# Autodesk Inventor assembly: Exoskeleton
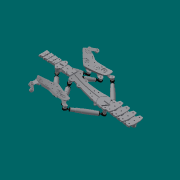
[picture p0: Inventor's stored thumbnail of the model, 180x180]
Saved by Autodesk Inventor 2015 SP1 (Build 190203100, 203)
## iProperties
Created: 2016-10-02
Part Number: Exoskeleton
Document SubType Name: Assembly
Designer: Val
Author: Val
## Documents named in this file (24)
- C:\Users\Val\Desktop\ExoGit\elysium-max-exoskeleton\src\Assemblies\Exoskeleton.iam
- C:\Users\Val\Desktop\ExoGit\elysium-max-exoskeleton\src\Assemblies\ChestDerived.iam
- C:\Users\Val\Desktop\ExoGit\elysium-max-exoskeleton\src\Assemblies\Spine.iam
- C:\Users\Val\Desktop\ExoGit\elysium-max-exoskeleton\src\Assemblies\Pelvis.iam
- C:\Users\Val\Desktop\ExoGit\elysium-max-exoskeleton\src\Assemblies\HipLeft.iam
- C:\Users\Val\Desktop\ExoGit\elysium-max-exoskeleton\src\Assemblies\HipRight.iam
- C:\Users\Val\Desktop\ExoGit\elysium-max-exoskeleton\src\Assemblies\ShoulderLeft.iam
- C:\Users\Val\Desktop\ExoGit\elysium-max-exoskeleton\src\Assemblies\ShoulderRight.iam
- C:\Users\Val\Desktop\ExoGit\elysium-max-exoskeleton\src\Assemblies\UpperArmLeft.iam
- C:\Users\Val\Desktop\ExoGit\elysium-max-exoskeleton\src\Assemblies\UpperArmRight.iam
- C:\Users\Val\Desktop\ExoGit\elysium-max-exoskeleton\src\Assemblies\ForearmLeft.iam
- C:\Users\Val\Desktop\ExoGit\elysium-max-exoskeleton\src\Assemblies\ForearmRight.iam
- C:\Users\Val\Desktop\ExoGit\elysium-max-exoskeleton\src\Assemblies\HandLeft.iam
- C:\Users\Val\Desktop\ExoGit\elysium-max-exoskeleton\src\Assemblies\HandRight.iam
- C:\Users\Val\Desktop\ExoGit\elysium-max-exoskeleton\src\Assemblies\LegLeft.iam
- C:\Users\Val\Desktop\ExoGit\elysium-max-exoskeleton\src\Assemblies\LegRight.iam
- C:\Users\Val\Desktop\ExoGit\elysium-max-exoskeleton\src\Assemblies\Pistons\PistonBackTop.iam
- C:\Users\Val\Desktop\ExoGit\elysium-max-exoskeleton\src\Assemblies\Pistons\PistonBackMiddle.iam
- C:\Users\Val\Desktop\ExoGit\elysium-max-exoskeleton\src\Assemblies\Pistons\PistonBackBottom.iam
- C:\Users\Val\Desktop\ExoGit\elysium-max-exoskeleton\src\Assemblies\Pistons\PistonTricep.iam
- C:\Users\Val\Desktop\ExoGit\elysium-max-exoskeleton\src\Assemblies\Pistons\PistonHipBack.iam
- C:\Users\Val\Desktop\ExoGit\elysium-max-exoskeleton\src\Assemblies\Pistons\PistonHipFront.iam
- C:\Users\Val\Desktop\ExoGit\elysium-max-exoskeleton\src\Assemblies\Pistons\PistonHipMiddle.iam
- C:\Users\Val\Desktop\ExoGit\elysium-max-exoskeleton\src\Assemblies\Pistons\PistonLeg.iam
## Components (31 placed, 23 different names)
1. ChestDerived:1 [sub-assembly] — Flush:1, Flush:2
2. Spine:1 [sub-assembly] — Mate:1, Angle:1, Mate:43, Mate:44, Mate:45, Mate:46, Mate:47, Mate:48
3. Pelvis:1 [sub-assembly] — Mate:35
4. HipLeft:1 [sub-assembly] — Mate:31, Mate:36, Mate:37
5. HipRight:1 [sub-assembly] — Mate:38, Mate:39, Mate:40
6. ShoulderLeft:1 [sub-assembly]
7. ShoulderRight:1 [sub-assembly]
8. UpperArmLeft:1 [sub-assembly] — Mate:2, Mate:3, Mate:20, Mate:21
9. UpperArmRight:1 [sub-assembly] — Mate:4, Mate:5, Mate:22, Mate:23
10. ForearmLeft:1 [sub-assembly] — Mate:2, Mate:3
11. ForearmRight:1 [sub-assembly] — Mate:4, Mate:5
12. HandLeft:1 [sub-assembly]
13. HandRight:1 [sub-assembly]
14. LegLeft:1 [sub-assembly] — Mate:41
15. LegRight:1 [sub-assembly] — Mate:42
16. PistonBackTop:1 [sub-assembly] — Mate:48
17. PistonBackTop:2 [sub-assembly] — Mate:45
18. PistonBackMiddle:1 [sub-assembly] — Mate:47
19. PistonBackMiddle:2 [sub-assembly] — Mate:44
20. PistonBackBottom:1 [sub-assembly] — Mate:46
21. PistonBackBottom:2 [sub-assembly] — Mate:43
22. PistonTricep:2 [sub-assembly] — Mate:20, Mate:21
23. PistonTricep:3 [sub-assembly] — Mate:22, Mate:23
24. PistonHipBack:1 [sub-assembly] — Mate:38
25. PistonHipFront:1 [sub-assembly] — Mate:40
26. PistonHipMiddle:1 [sub-assembly] — Mate:39
27. PistonHipBack:2 [sub-assembly] — Mate:37
28. PistonHipFront:2 [sub-assembly] — Mate:31, Mate:35
29. PistonHipMiddle:2 [sub-assembly] — Mate:36
30. PistonLeg:1 [sub-assembly] — Mate:41
31. PistonLeg:2 [sub-assembly] — Mate:42
## Relationships (28: Mate 24, Flush 2, Symmetry 1, Angle 1)
- Flush:1: ChestDerived:1
- Flush:2: ChestDerived:1
- Symmetry:1
- Mate:1: Spine:1
- Angle:1 (0 deg): Spine:1
- Mate:2: UpperArmLeft:1 ↔ ForearmLeft:1
- Mate:3: UpperArmLeft:1 ↔ ForearmLeft:1
- Mate:4: UpperArmRight:1 ↔ ForearmRight:1
- Mate:5: UpperArmRight:1 ↔ ForearmRight:1
- Mate:20: UpperArmLeft:1 ↔ PistonTricep:2
- Mate:21: UpperArmLeft:1 ↔ PistonTricep:2
- Mate:22: UpperArmRight:1 ↔ PistonTricep:3
- Mate:23: UpperArmRight:1 ↔ PistonTricep:3
- Mate:31: HipLeft:1 ↔ PistonHipFront:2
- Mate:35: Pelvis:1 ↔ PistonHipFront:2
- Mate:36: HipLeft:1 ↔ PistonHipMiddle:2
- Mate:37: HipLeft:1 ↔ PistonHipBack:2
- Mate:38: HipRight:1 ↔ PistonHipBack:1
- Mate:39: HipRight:1 ↔ PistonHipMiddle:1
- Mate:40: HipRight:1 ↔ PistonHipFront:1
- Mate:41: LegLeft:1 ↔ PistonLeg:1
- Mate:42: LegRight:1 ↔ PistonLeg:2
- Mate:43: Spine:1 ↔ PistonBackBottom:2
- Mate:44: Spine:1 ↔ PistonBackMiddle:2
- Mate:45: Spine:1 ↔ PistonBackTop:2
- Mate:46: Spine:1 ↔ PistonBackBottom:1
- Mate:47: Spine:1 ↔ PistonBackMiddle:1
- Mate:48: Spine:1 ↔ PistonBackTop:1
